# Autodesk Inventor assembly: Assembly Ficha de Exercício 9
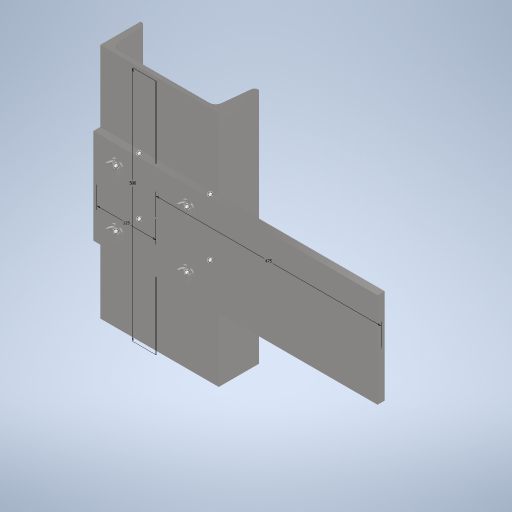
[picture p0: Inventor's stored thumbnail of the model, 512x512]
Saved by Autodesk Inventor 2024 (Build 280153000, 153)
## iProperties
Created: 2024-04-29
Part Number: Assembly Ficha de Exercício 9
Document SubType Name: Assembly
Designer: Pedro
_SolveAssemblyDoc: Frame Generator Solve Assembly
_Version: 25.0.0
Author: Pedro
## Documents named in this file (6)
- C:\Users\Pedro\Desktop\Autodesk Inbentor\Aula 10\Assembly Ficha de Exercício 9.iam
- C:\Users\Pedro\Desktop\Autodesk Inbentor\Aula 10\Exercício 9.ipt
- C:\Users\Pedro\Desktop\Autodesk Inbentor\Aula 10\Assembly Ficha de Exercício 9\Frame\Frame 1714380559291.iam
- C:\Users\Pedro\Documents\Inventor\Content Center Files\R2024\en-US\ISO 7089\ISO 7089 - 16 - 140 HV(1).ipt
- C:\Users\Pedro\Documents\Inventor\Content Center Files\R2024\en-US\ISO 4014(2)\ISO 4014 - M16 x 65 - ISO.ipt
- C:\Users\Pedro\Documents\Inventor\Content Center Files\R2024\en-US\ISO 4032(2)\ISO 4032 - M16 - ISO.ipt
## Components (18 placed, 5 different names)
1. Exercício 9:1
2. Frame 1714380559291:1 [sub-assembly] — Mate:17, Mate:18, Mate:19, Mate:20, Mate:21, Mate:22, Mate:23, Mate:24, Mate:25, Mate:26, Mate:27, Mate:28, Mate:29, Mate:30, Mate:31, Mate:32
3. ISO 7089 16:1 — Mate:29, Mate:30, Insert:12
4. ISO 4014 M16 x 65:1 — Insert:12
5. ISO 4032 M16:1 — Insert:13
6. ISO 7089 16:2 — Mate:17, Mate:18, Insert:6
7. ISO 4014 M16 x 65:2 — Insert:6
8. ISO 4032 M16:2 — Insert:7
9. ISO 7089 16:3 — Mate:21, Mate:22, Insert:8
10. ISO 4014 M16 x 65:3 — Insert:8
11. ISO 4032 M16:3 — Insert:9
12. ISO 7089 16:4 — Mate:31, Mate:32, Insert:13
13. ISO 7089 16:5 — Mate:19, Mate:20, Insert:7
14. ISO 7089 16:6 — Mate:23, Mate:24, Insert:9
15. ISO 7089 16:7 — Mate:25, Mate:26, Insert:10
16. ISO 4014 M16 x 65:4 — Insert:10
17. ISO 7089 16:8 — Mate:27, Mate:28, Insert:11
18. ISO 4032 M16:4 — Insert:11
## Relationships (24: Mate 16, Insert 8)
- Mate:17: Frame 1714380559291:1 ↔ ISO 7089 16:2
- Mate:18: Frame 1714380559291:1 ↔ ISO 7089 16:2
- Insert:6: ISO 7089 16:2 ↔ ISO 4014 M16 x 65:2
- Mate:19: Frame 1714380559291:1 ↔ ISO 7089 16:5
- Mate:20: Frame 1714380559291:1 ↔ ISO 7089 16:5
- Insert:7: ISO 4032 M16:2 ↔ ISO 7089 16:5
- Mate:21: Frame 1714380559291:1 ↔ ISO 7089 16:3
- Mate:22: Frame 1714380559291:1 ↔ ISO 7089 16:3
- Insert:8: ISO 7089 16:3 ↔ ISO 4014 M16 x 65:3
- Mate:23: Frame 1714380559291:1 ↔ ISO 7089 16:6
- Mate:24: Frame 1714380559291:1 ↔ ISO 7089 16:6
- Insert:9: ISO 4032 M16:3 ↔ ISO 7089 16:6
- Mate:25: Frame 1714380559291:1 ↔ ISO 7089 16:7
- Mate:26: Frame 1714380559291:1 ↔ ISO 7089 16:7
- Insert:10: ISO 7089 16:7 ↔ ISO 4014 M16 x 65:4
- Mate:27: Frame 1714380559291:1 ↔ ISO 7089 16:8
- Mate:28: Frame 1714380559291:1 ↔ ISO 7089 16:8
- Insert:11: ISO 7089 16:8 ↔ ISO 4032 M16:4
- Mate:29: Frame 1714380559291:1 ↔ ISO 7089 16:1
- Mate:30: Frame 1714380559291:1 ↔ ISO 7089 16:1
- Insert:12: ISO 7089 16:1 ↔ ISO 4014 M16 x 65:1
- Mate:31: Frame 1714380559291:1 ↔ ISO 7089 16:4
- Mate:32: Frame 1714380559291:1 ↔ ISO 7089 16:4
- Insert:13: ISO 4032 M16:1 ↔ ISO 7089 16:4
